# Autodesk Inventor assembly: Spin3_Enclosure
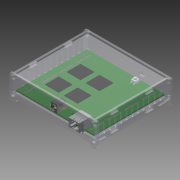
[picture p0: Inventor's stored thumbnail of the model, 180x180]
Saved by Autodesk Inventor 2015 SP1 (Build 190203100, 203)
## iProperties
Created: 2015-01-22
Part Number: Spin3_Enclosure
Document SubType Name: Assembly
Designer: Patrick
Author: Patrick
## Documents named in this file (7)
- C:\Users\Patrick\CAD\Spin3 Enclosure\Spin3_Enclosure.iam
- C:\Users\Patrick\CAD\Spin3 Enclosure\PCB_Components.iam
- C:\Users\Patrick\CAD\Spin3 Enclosure\BottomPanel.ipt
- C:\Users\Patrick\CAD\Spin3 Enclosure\FrontPanel.ipt
- C:\Users\Patrick\CAD\Spin3 Enclosure\SidePanel.ipt
- C:\Users\Patrick\CAD\Spin3 Enclosure\BackPanel.ipt
- C:\Users\Patrick\CAD\Spin3 Enclosure\TopPanel.ipt
## Components (7 placed, 6 different names)
1. PCB_Components:1 [sub-assembly] — Rigid:11
2. BottomPanel:1 — Rigid:6, Rigid:11
3. FrontPanel:1 — Rigid:7, Rigid:9
4. SidePanel:1 — Rigid:9
5. SidePanel:2 — Rigid:6, Rigid:7, Rigid:8, Rigid:10
6. BackPanel:1 — Rigid:8
7. TopPanel:1 — Rigid:10
## Relationships (6: WeldJoint 6)
- Rigid:6 [WeldJoint]: BottomPanel:1 ↔ SidePanel:2
- Rigid:7 [WeldJoint]: FrontPanel:1 ↔ SidePanel:2
- Rigid:8 [WeldJoint]: SidePanel:2 ↔ BackPanel:1
- Rigid:9 [WeldJoint]: FrontPanel:1 ↔ SidePanel:1
- Rigid:10 [WeldJoint]: SidePanel:2 ↔ TopPanel:1
- Rigid:11 [WeldJoint] (-3 mm): PCB_Components:1 ↔ BottomPanel:1
